# Autodesk Inventor assembly: DemonstratorUITräger
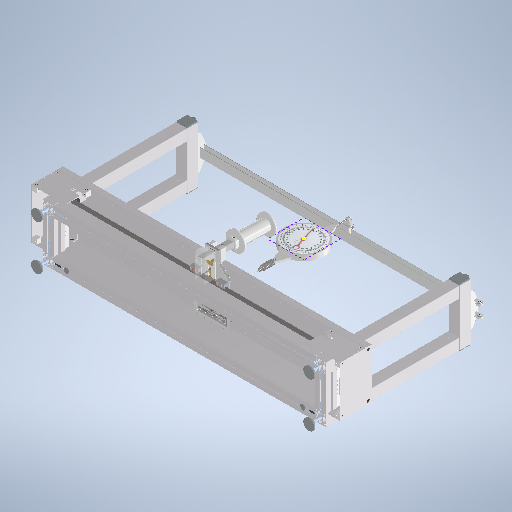
[picture p0: Inventor's stored thumbnail of the model, 512x512]
Saved by Autodesk Inventor 2025 (Build 290162010, 162A)
## iProperties
Created: 2024-11-07
Part Number: DemonstratorUITräger
Document SubType Name: Assembly
Designer: Admin
Mass: 19237.8 g
Surface Area: 46696.5 cm^2
Volume: 6430.49 cm^3
Density: 2.99166 g/cm^3
dummerWinkel: 1.5
Author: Admin
## Documents named in this file (39)
- C:\Users\Admin\GIT\HDVKBM\CAD\Krandemonstrator\DemonstratorUITräger.iam
- C:\Users\Admin\GIT\HDVKBM\CAD\Krandemonstrator\Träger.ipt
- C:\Users\Admin\GIT\HDVKBM\CAD\Krandemonstrator\Katze.iam
- C:\Users\Admin\GIT\HDVKBM\CAD\Krandemonstrator\UmlenkrolleHalterEinfach.iam
- C:\Users\Admin\GIT\HDVKBM\CAD\Krandemonstrator\SeilStange1m.ipt
- C:\Users\Admin\GIT\HDVKBM\CAD\Krandemonstrator\RollenhalterU.ipt
- C:\Users\Admin\GIT\HDVKBM\CAD\Krandemonstrator\UmlenkrolleHalterDoppelt.iam
- C:\Users\Admin\GIT\HDVKBM\CAD\Krandemonstrator\SeilatrappeHalter.ipt
- C:\Users\Admin\GIT\HDVKBM\CAD\Krandemonstrator\UmlenkrolleHalterDoppeltAngle.iam
- C:\Users\Admin\GIT\HDVKBM\CAD\Krandemonstrator\UmlenkrolleHalterEinfachAngle.iam
- C:\Users\Admin\GIT\HDVKBM\CAD\Krandemonstrator\UmlenkrolleHalterEinfachAngleB.iam
- C:\Users\Admin\GIT\HDVKBM\CAD\Krandemonstrator\seilatrappeHalterMini.ipt
- C:\Users\Admin\GIT\HDVKBM\CAD\Krandemonstrator\WS_10_40_930_2\WS_10_40_930_2.iam
- C:\Users\Admin\GIT\HDVKBM\CAD\Krandemonstrator\Frame.iam
- C:\Users\Admin\GIT\HDVKBM\CAD\Krandemonstrator\item_42006_nutenstein-8-st-m4-verzi__high\item_42006_nutenstein-8-st-m4-verzi__high.ipt
- C:\Users\Admin\GIT\HDVKBM\CAD\Krandemonstrator\item_2623_nutenstein-8-st-m6-verzi__high\item_2623_nutenstein-8-st-m6-verzi__high.ipt
- C:\Users\Admin\GIT\HDVKBM\CAD\Krandemonstrator\Zugfeder11.ipt
- C:\Users\Admin\GIT\HDVKBM\CAD\Krandemonstrator\Bedienhebel.iam
- C:\Users\Admin\GIT\HDVKBM\CAD\Krandemonstrator\SeilStange3cm.ipt
- C:\Users\Admin\GIT\HDVKBM\CAD\Krandemonstrator\waage.ipt
- C:\Users\Admin\GIT\HDVKBM\CAD\Krandemonstrator\verkleidungBremse.ipt
- C:\Users\Admin\Documents\Inventor\Content Center Files\R2025\de-DE\DIN EN ISO 7089\DIN EN ISO 7089 -  5.ipt
- C:\Users\Admin\Documents\Inventor\Content Center Files\R2025\de-DE\DIN 933\DIN 933 - M5  x 8.ipt
- C:\Users\Admin\GIT\HDVKBM\CAD\Krandemonstrator\item_42005_nutenstein-8-st-m5-verzi__high\item_42005_nutenstein-8-st-m5-verzi__high.ipt
- C:\Users\Admin\Documents\Inventor\Content Center Files\R2025\de-DE\DIN 933\DIN 933 - M5  x 18.ipt
- C:\Users\Admin\GIT\HDVKBM\CAD\Krandemonstrator\Schlitten.iam
- C:\Users\Admin\GIT\HDVKBM\CAD\Krandemonstrator\SeilStange447mm.ipt
- C:\Users\Admin\Documents\Inventor\Content Center Files\R2025\de-DE\ISO 4032(1)\ISO 4032 - M4DIN EN.ipt
- C:\Users\Admin\Documents\Inventor\Content Center Files\R2025\de-DE\DIN EN ISO 4026\DIN EN ISO 4026 - M4 x 8.ipt
- C:\Users\Admin\Documents\Inventor\Content Center Files\R2025\de-DE\ISO 2009(1)\ISO 2009 - M2 x 4 - DIN EN 2.ipt
- C:\Users\Admin\Documents\Inventor\Content Center Files\R2025\de-DE\ISO 10642(2)\ISO 10642  - M4  x  25.ipt
- C:\Users\Admin\Documents\Inventor\Content Center Files\R2025\de-DE\ISO 10642(2)\ISO 10642  - M6  x  16.ipt
- C:\Users\Admin\Documents\Inventor\Content Center Files\R2025\de-DE\ISO 10642(2)\ISO 10642  - M3  x  16.ipt
- C:\Users\Admin\Documents\Inventor\Content Center Files\R2025\de-DE\ISO 10642(2)\ISO 10642  - M3  x  25.ipt
- C:\Users\Admin\Documents\Inventor\Content Center Files\R2025\de-DE\ISO 2009(1)\ISO 2009 - M2 x 6 - DIN EN 4.ipt
- C:\Users\Admin\Documents\Inventor\Content Center Files\R2025\de-DE\ISO 10642(2)\ISO 10642  - M4  x  30.ipt
- C:\Users\Admin\GIT\HDVKBM\CAD\Krandemonstrator\Platte Scharfe Ecken (mm) 150 x 30 x 8 - UITräger.ipt
- C:\Users\Admin\GIT\HDVKBM\CAD\Krandemonstrator\MontageAufnahmeLO-LH_UI.ipt
- C:\Users\Admin\GIT\HDVKBM\CAD\Krandemonstrator\MontageAufnahmeLO_UI.ipt
## Components (139 placed, 40 different names)
1. Katze:1 [sub-assembly] — KatzeLagerHO, KatzeLagerVV, KatzeGewindeSeilStumpfVL, KatzeSeilStumpfHL, KatzeSeilStumpfVR, KatzeSeilStumpfHR, Zylindrisch:83
2. Frame:1 [sub-assembly] — Verschiebbar:90, Verschiebbar:89, Starr:89, Starr:124, Starr:134, Starr:136, Planar:60, Planar:61
3. DIN EN ISO 7089 5:1
4. DIN EN ISO 7089 5:2
5. DIN EN ISO 7089 5:3
6. DIN EN ISO 7089 5:4
7. DIN 933 - ersetzt durch DIN EN 24017 M5  x 8:1
8. DIN 933 - ersetzt durch DIN EN 24017 M5  x 8:2 — Zylindrisch:109
9. DIN 933 - ersetzt durch DIN EN 24017 M5  x 8:3
10. DIN 933 - ersetzt durch DIN EN 24017 M5  x 8:4 — Zylindrisch:110
11. Platte Scharfe Ecken (mm) 150 x 30 x 8 - UITräger:2 — Starr:136, Einfügen:8, Zylindrisch:110
12. Platte Scharfe Ecken (mm) 150 x 30 x 8 - UITräger:1 — Starr:134, Zylindrisch:109, Planar:57
13. DIN 933 - ersetzt durch DIN EN 24017 M5  x 18:2
14. DIN 933 - ersetzt durch DIN EN 24017 M5  x 18:3
15. DIN 933 - ersetzt durch DIN EN 24017 M5  x 18:4
16. DIN 933 - ersetzt durch DIN EN 24017 M5  x 18:1 — Einfügen:8
17. DIN EN ISO 10642 M3  x  25:1
18. DIN EN ISO 10642 M3  x  25:2
19. DIN EN ISO 10642 M3  x  25:3
20. DIN EN ISO 10642 M3  x  25:4
21. DIN EN ISO 10642 M3  x  16:1
22. DIN EN ISO 10642 M3  x  16:2
23. DIN EN ISO 10642 M3  x  16:3
24. DIN EN ISO 10642 M3  x  16:4
25. MontageAufnahmeLO-LH_UI:1 — SeilrolleORHplan, Starr:137
26. MontageAufnahmeLO_UI:1 — SeilrolleORVplan, Starr:138
27. MontageAufnahmeLOV:1 — SeilrolleOLVAuflage, Starr:140
28. MontageAufnahmeLOH:1 — SeilrolleOLHAuflage, Starr:139
29. item_42005_nutenstein-8-st-m5-verzi__high:1
30. item_42005_nutenstein-8-st-m5-verzi__high:2
31. item_42005_nutenstein-8-st-m5-verzi__high:4
32. item_42005_nutenstein-8-st-m5-verzi__high:3
33. Träger:1 — KatzeLagerHO, KatzeLagerVV, Starr:137, Starr:138, Starr:139, Starr:140, Planar:57
34. Bedienhebel:1 [sub-assembly] — Kugelförmig:1, Kugelförmig:3, Planar:58
35. DIN EN ISO 10642 M4  x  25:1
36. DIN EN ISO 10642 M4  x  25:2 — Zylindrisch:142
37. DIN EN ISO 10642 M4  x  25:3 — Zylindrisch:143
38. DIN EN ISO 10642 M4  x  25:4
39. verkleidungBremse:1 — Planar:59
40. DIN EN ISO 2009 M2 x 4:1
41. DIN EN ISO 2009 M2 x 4:2
42. DIN EN ISO 2009 M2 x 4:3
43. DIN EN ISO 2009 M2 x 4:4
44. Schlitten:1 [sub-assembly] — Zylindrisch:111, Zylindrisch:112, Zylindrisch:142, Zylindrisch:143, Planar:58, Planar:59, Verschiebbar:1, Kugelförmig:4, Kugelförmig:5
45. lastseil — Zylindrisch:83, Starr:117, Verschiebbar:1
46. Zugfeder1:1 — Starr:118
47. waage:1 — Starr:117, Starr:118
48. SeilStange3cm:5 — Zylindrisch:146, Kugelförmig:3
49. SeilStange3cm:6 — Zylindrisch:146, Kugelförmig:5
50. SeilStange3cm:7 — Starr:122
51. SeilStange3cm:8 — Starr:122, Starr:123
52. SeilStange3cm:2 — Zylindrisch:108, Kugelförmig:4
53. SeilStange3cm:1 — Kugelförmig:1, Zylindrisch:108, Starr:123
54. seilatrappeHalterMini:3 — SeilAtrappeHalterMini3, SeilAtrappeHalterMini3Seil
55. seilatrappeHalterMini:4 — SeilAtrappeHalterMini4, SeilAtrappeHalterMini4Seil
56. seilatrappeHalterMini:1 — SeilAtrappeHalterMini1, SeilAtrappeHalterMini1Seil
57. seilatrappeHalterMini:2 — SeilAtrappeHalterMini2, SeilAtrappeHalterMini2Seil
58. SeilatrappeHalter:1 — SeilAtrappeHalterSeilA, SeilAtrappeHalterSeilB, Starr:124
59. SeilStange1m:16 — SeilrolleULMVsld, SeilAtrappeHalterMini3Seil
60. SeilStange1m:17 — SeilrolleULMHsld, SeilAtrappeHalterMini4Seil
61. SeilStange1m:18 — SeilAtrappeHalterMini1Seil, SeilrolleORVver, SeilrolleURMVver
62. SeilStange1m:19 — SeilAtrappeHalterMini2Seil, SeilrolleORHver, SeilrolleURMHver
63. SeilStange1m:13 — SeilrolleURHsld
64. SeilStange1m:12 — SeilrolleURVsld
65. SeilStange1m:1 — KatzeGewindeSeilStumpfVL, SeilrolleOLVhor
66. SeilStange1m:3 — SeilrolleOLHhor, KatzeSeilStumpfHL
67. SeilStange1m:4 — SeilrolleORHhor, KatzeSeilStumpfHR
68. SeilStange1m:5 — SeilrolleORVhor, KatzeSeilStumpfVR
69. SeilStange1m:8 — SeilAtrappeHalterSeilB, SeilrolleOLHver, SeilrolleULHver
70. SeilStange1m:9 — SeilAtrappeHalterSeilA, SeilrolleOLVver, SeilrolleULVver
71. SeilStange1m:10 — Zylindrisch:15, SeilrolleULHhor, SeilrolleURHhor
72. SeilStange1m:11 — Zylindrisch:16, SeilrolleULVhor, SeilrolleURVhor
73. SeilStange1m:14 — SeilAtrappeRollenhalterSeilB, SeilrolleULMHhor, SeilrolleURMHhor
74. SeilStange1m:15 — SeilAtrappeRollenhalterSeilA, SeilrolleULMVhor, SeilrolleURMVhor
75. item_2623_nutenstein-8-st-m6-verzi__high:1 — Starr:90
76. item_2623_nutenstein-8-st-m6-verzi__high:2 — Starr:91
77. item_2623_nutenstein-8-st-m6-verzi__high:3 — Starr:96
78. item_2623_nutenstein-8-st-m6-verzi__high:4 — Starr:92
79. item_2623_nutenstein-8-st-m6-verzi__high:5 — Starr:93
80. item_2623_nutenstein-8-st-m6-verzi__high:6 — Starr:94
81. item_2623_nutenstein-8-st-m6-verzi__high:7 — Starr:95
82. item_2623_nutenstein-8-st-m6-verzi__high:8 — Starr:97
83. DIN EN ISO 10642 M6  x  16:1 — Starr:90, Starr:105
84. DIN EN ISO 10642 M6  x  16:2 — Starr:91, Starr:104
85. DIN EN ISO 10642 M6  x  16:3 — Starr:93, Starr:102
86. DIN EN ISO 10642 M6  x  16:4 — Starr:92, Starr:103
87. DIN EN ISO 10642 M6  x  16:5 — Starr:97, Starr:98
88. DIN EN ISO 10642 M6  x  16:6 — Starr:96, Starr:99
89. DIN EN ISO 10642 M6  x  16:7 — Starr:95, Starr:100
90. DIN EN ISO 10642 M6  x  16:8 — Starr:94, Starr:101
91. WS_10_40_930_2:1 [sub-assembly] — Starr:89, Zylindrisch:111, Zylindrisch:112, Starr:98, Starr:99, Starr:100, Starr:101, Starr:105, Starr:104, Starr:102, Starr:103
92. DIN EN ISO 2009 M2 x 6:1
93. DIN EN ISO 2009 M2 x 6:2
94. UmlenkrolleHalterEinfach:1 [sub-assembly] — SeilrolleOLVAuflage, SeilrolleOLVhor, SeilrolleOLVver
95. DIN EN ISO 2009 M2 x 6:3
96. DIN EN ISO 2009 M2 x 6:4
97. UmlenkrolleHalterEinfach:2 [sub-assembly] — SeilrolleOLHAuflage, SeilrolleOLHhor, SeilrolleOLHver
98. DIN EN 24032 M4:1
99. DIN EN 24032 M4:2
100. DIN EN 24032 M4:3
101. DIN EN 24032 M4:4
102. DIN EN ISO 4026 M4 x 8:1
103. DIN EN ISO 4026 M4 x 8:2
104. DIN EN ISO 4026 M4 x 8:3
105. DIN EN ISO 4026 M4 x 8:4
106. UmlenkrolleHalterEinfachAngle:1 [sub-assembly] — SeilrolleORVplan, SeilrolleORVhor, SeilrolleORVver, SeilAtrappeHalterMini1
107. DIN EN ISO 2009 M2 x 6:5
108. DIN EN ISO 2009 M2 x 6:6
109. DIN EN ISO 2009 M2 x 6:7
110. DIN EN ISO 2009 M2 x 6:8
111. UmlenkrolleHalterEinfachAngleB:1 [sub-assembly] — SeilrolleORHplan, SeilAtrappeHalterMini2, SeilrolleORHhor, SeilrolleORHver
112. RollenhalterU:1 — Planar:24, Planar:25, Planar:40, Zylindrisch:15, Zylindrisch:16, Starr:84, Starr:85, Verschiebbar:89, Planar:60
113. DIN EN ISO 10642 M4  x  30:1
114. DIN EN ISO 10642 M4  x  30:2
115. UmlenkrolleHalterDoppelt:1 [sub-assembly] — Planar:24, SeilrolleULMHhor, SeilrolleULMVhor, SeilrolleULMHsld, SeilrolleULMVsld, SeilAtrappeHalterMini3, SeilAtrappeHalterMini4
116. UmlenkrolleHalterEinfach:3 [sub-assembly] — Planar:25, SeilrolleULVver, SeilrolleULVhor
117. UmlenkrolleHalterEinfach:4 [sub-assembly] — Planar:40, SeilrolleULHver, SeilrolleULHhor
118. DIN EN ISO 2009 M2 x 6:9
119. DIN EN ISO 2009 M2 x 6:10
120. DIN EN ISO 2009 M2 x 6:11
121. DIN EN ISO 2009 M2 x 6:12
122. DIN EN ISO 2009 M2 x 6:13
123. item_42006_nutenstein-8-st-m4-verzi__high:1 — Starr:85
124. item_42006_nutenstein-8-st-m4-verzi__high:2 — Starr:84
125. DIN EN ISO 2009 M2 x 6:14
126. UmlenkrolleHalterEinfach:5 [sub-assembly] — Planar:42, SeilrolleURVhor, SeilrolleURVsld
127. UmlenkrolleHalterEinfach:6 [sub-assembly] — Planar:43, SeilrolleURHhor, SeilrolleURHsld
128. UmlenkrolleHalterDoppeltAngle:1 [sub-assembly] — Planar:54, SeilrolleURMHhor, SeilrolleURMVhor, SeilrolleURMVver, SeilrolleURMHver
129. DIN EN ISO 2009 M2 x 6:15
130. DIN EN ISO 2009 M2 x 6:16
131. DIN EN ISO 2009 M2 x 6:17
132. DIN EN ISO 2009 M2 x 6:18
133. DIN EN ISO 2009 M2 x 6:19
134. DIN EN ISO 2009 M2 x 6:20
135. RollenhalterU:2 — Planar:42, Planar:43, Planar:54, SeilAtrappeRollenhalterSeilB, SeilAtrappeRollenhalterSeilA, Verschiebbar:90, Starr:86, Starr:87, Planar:61
136. DIN EN ISO 10642 M4  x  30:3
137. item_42006_nutenstein-8-st-m4-verzi__high:3 — Starr:87
138. item_42006_nutenstein-8-st-m4-verzi__high:4 — Starr:86
139. DIN EN ISO 10642 M4  x  30:4
## Relationships (189: WeldJoint 74, CylindricalJoint 41, RelateRotateTranslate 24, Mate 18, PlanarJoint 17, Insert 8, BallJoint 4, TranslationJoint 3)
- KatzeLagerHO [PlanarJoint] (0.05 mm): Katze:1 ↔ Träger:1
- KatzeLagerVV [PlanarJoint] (0.05 mm): Katze:1 ↔ Träger:1
- [WeldJoint]: Katze:1 ↔ DIN EN 24032 M4:2
- [WeldJoint]: Katze:1 ↔ DIN EN 24032 M4:4
- [WeldJoint]: Katze:1 ↔ DIN EN 24032 M4:1
- [WeldJoint]: Katze:1 ↔ DIN EN 24032 M4:3
- KatzeGewindeSeilStumpfVL [WeldJoint]: Katze:1 ↔ SeilStange1m:1
- [WeldJoint]: Katze:1 ↔ DIN EN ISO 4026 M4 x 8:4
- [WeldJoint]: Katze:1 ↔ DIN EN ISO 4026 M4 x 8:2
- [WeldJoint]: Katze:1 ↔ DIN EN ISO 4026 M4 x 8:1
- [WeldJoint]: Katze:1 ↔ DIN EN ISO 4026 M4 x 8:3
- KatzeSeilStumpfHL [WeldJoint]: Katze:1 ↔ SeilStange1m:3
- KatzeSeilStumpfVR [WeldJoint]: Katze:1 ↔ SeilStange1m:5
- KatzeSeilStumpfHR [WeldJoint]: Katze:1 ↔ SeilStange1m:4
- [WeldJoint]: DIN EN ISO 2009 M2 x 6:2 ↔ UmlenkrolleHalterEinfach:1
- [WeldJoint]: DIN EN ISO 2009 M2 x 6:1 ↔ UmlenkrolleHalterEinfach:1
- SeilrolleOLVAuflage [PlanarJoint]: MontageAufnahmeLOV:1 ↔ UmlenkrolleHalterEinfach:1
- [CylindricalJoint]: MontageAufnahmeLOV:1 ↔ DIN EN ISO 2009 M2 x 6:1
- [CylindricalJoint]: MontageAufnahmeLOV:1 ↔ DIN EN ISO 2009 M2 x 6:2
- SeilrolleOLVhor [RelateRotateTranslate] (9 mm): SeilStange1m:1 ↔ UmlenkrolleHalterEinfach:1
- SeilrolleOLVver [RelateRotateTranslate] (9 mm): SeilStange1m:9 ↔ UmlenkrolleHalterEinfach:1
- [WeldJoint]: DIN EN ISO 2009 M2 x 6:3 ↔ UmlenkrolleHalterEinfach:2
- [WeldJoint]: DIN EN ISO 2009 M2 x 6:4 ↔ UmlenkrolleHalterEinfach:2
- SeilrolleOLHAuflage [PlanarJoint]: MontageAufnahmeLOH:1 ↔ UmlenkrolleHalterEinfach:2
- [CylindricalJoint]: MontageAufnahmeLOH:1 ↔ DIN EN ISO 2009 M2 x 6:3
- [CylindricalJoint]: MontageAufnahmeLOH:1 ↔ DIN EN ISO 2009 M2 x 6:4
- SeilrolleOLHhor [RelateRotateTranslate] (9 mm): SeilStange1m:3 ↔ UmlenkrolleHalterEinfach:2
- SeilrolleOLHver [RelateRotateTranslate] (9 mm): SeilStange1m:8 ↔ UmlenkrolleHalterEinfach:2
- Planar:24: RollenhalterU:1 ↔ UmlenkrolleHalterDoppelt:1
- [WeldJoint]: UmlenkrolleHalterDoppelt:1 ↔ DIN EN ISO 2009 M2 x 6:12
- [WeldJoint]: UmlenkrolleHalterDoppelt:1 ↔ DIN EN ISO 2009 M2 x 6:11
- [CylindricalJoint]: RollenhalterU:1 ↔ DIN EN ISO 2009 M2 x 6:12
- [CylindricalJoint]: RollenhalterU:1 ↔ DIN EN ISO 2009 M2 x 6:11
- [WeldJoint]: UmlenkrolleHalterEinfach:3 ↔ DIN EN ISO 2009 M2 x 6:13
- [WeldJoint]: UmlenkrolleHalterEinfach:3 ↔ DIN EN ISO 2009 M2 x 6:14
- Planar:25: RollenhalterU:1 ↔ UmlenkrolleHalterEinfach:3
- [CylindricalJoint]: RollenhalterU:1 ↔ DIN EN ISO 2009 M2 x 6:14
- [CylindricalJoint]: RollenhalterU:1 ↔ DIN EN ISO 2009 M2 x 6:13
- [WeldJoint]: UmlenkrolleHalterEinfach:4 ↔ DIN EN ISO 2009 M2 x 6:10
- [WeldJoint]: UmlenkrolleHalterEinfach:4 ↔ DIN EN ISO 2009 M2 x 6:9
- Planar:40: RollenhalterU:1 ↔ UmlenkrolleHalterEinfach:4
- [CylindricalJoint]: RollenhalterU:1 ↔ DIN EN ISO 2009 M2 x 6:9
- [CylindricalJoint]: RollenhalterU:1 ↔ DIN EN ISO 2009 M2 x 6:10
- SeilAtrappeHalterSeilA [CylindricalJoint]: SeilatrappeHalter:1 ↔ SeilStange1m:9
- SeilAtrappeHalterSeilB [CylindricalJoint]: SeilatrappeHalter:1 ↔ SeilStange1m:8
- Zylindrisch:15 [CylindricalJoint]: SeilStange1m:10 ↔ RollenhalterU:1
- Zylindrisch:16 [CylindricalJoint]: SeilStange1m:11 ↔ RollenhalterU:1
- SeilrolleULVver [RelateRotateTranslate] (9 mm): SeilStange1m:9 ↔ UmlenkrolleHalterEinfach:3
- SeilrolleULHver [RelateRotateTranslate] (9 mm): SeilStange1m:8 ↔ UmlenkrolleHalterEinfach:4
- SeilrolleULVhor [RelateRotateTranslate] (9 mm): SeilStange1m:11 ↔ UmlenkrolleHalterEinfach:3
- SeilrolleULHhor [RelateRotateTranslate] (9 mm): SeilStange1m:10 ↔ UmlenkrolleHalterEinfach:4
- [CylindricalJoint]: DIN EN ISO 2009 M2 x 6:19 ↔ RollenhalterU:2
- [CylindricalJoint]: DIN EN ISO 2009 M2 x 6:18 ↔ RollenhalterU:2
- [WeldJoint]: UmlenkrolleHalterEinfach:5 ↔ DIN EN ISO 2009 M2 x 6:17
- [WeldJoint]: UmlenkrolleHalterEinfach:5 ↔ DIN EN ISO 2009 M2 x 6:20
- Planar:42: UmlenkrolleHalterEinfach:5 ↔ RollenhalterU:2
- [CylindricalJoint]: DIN EN ISO 2009 M2 x 6:20 ↔ RollenhalterU:2
- [CylindricalJoint]: DIN EN ISO 2009 M2 x 6:17 ↔ RollenhalterU:2
- [WeldJoint]: UmlenkrolleHalterEinfach:6 ↔ DIN EN ISO 2009 M2 x 6:16
- [WeldJoint]: UmlenkrolleHalterEinfach:6 ↔ DIN EN ISO 2009 M2 x 6:15
- Planar:43: UmlenkrolleHalterEinfach:6 ↔ RollenhalterU:2
- [CylindricalJoint]: DIN EN ISO 2009 M2 x 6:16 ↔ RollenhalterU:2
- [CylindricalJoint]: DIN EN ISO 2009 M2 x 6:15 ↔ RollenhalterU:2
- SeilrolleURHhor [RelateRotateTranslate] (9 mm): SeilStange1m:10 ↔ UmlenkrolleHalterEinfach:6
- SeilrolleURVhor [RelateRotateTranslate] (9 mm): SeilStange1m:11 ↔ UmlenkrolleHalterEinfach:5
- SeilrolleURVsld [RelateRotateTranslate] (9 mm): SeilStange1m:12 ↔ UmlenkrolleHalterEinfach:5
- SeilrolleURHsld [RelateRotateTranslate] (9 mm): SeilStange1m:13 ↔ UmlenkrolleHalterEinfach:6
- Planar:54: UmlenkrolleHalterDoppeltAngle:1 ↔ RollenhalterU:2
- [WeldJoint]: UmlenkrolleHalterDoppeltAngle:1 ↔ DIN EN ISO 2009 M2 x 6:18
- [WeldJoint]: UmlenkrolleHalterDoppeltAngle:1 ↔ DIN EN ISO 2009 M2 x 6:19
- [WeldJoint]: UmlenkrolleHalterEinfachAngle:1 ↔ DIN EN ISO 2009 M2 x 6:6
- [WeldJoint]: UmlenkrolleHalterEinfachAngle:1 ↔ DIN EN ISO 2009 M2 x 6:5
- SeilrolleORVplan [PlanarJoint]: MontageAufnahmeLO_UI:1 ↔ UmlenkrolleHalterEinfachAngle:1
- [CylindricalJoint]: MontageAufnahmeLO_UI:1 ↔ DIN EN ISO 2009 M2 x 6:6
- [CylindricalJoint]: MontageAufnahmeLO_UI:1 ↔ DIN EN ISO 2009 M2 x 6:5
- [CylindricalJoint]: MontageAufnahmeLO-LH_UI:1 ↔ DIN EN ISO 2009 M2 x 6:8
- [CylindricalJoint]: MontageAufnahmeLO-LH_UI:1 ↔ DIN EN ISO 2009 M2 x 6:7
- SeilrolleORHplan [PlanarJoint]: MontageAufnahmeLO-LH_UI:1 ↔ UmlenkrolleHalterEinfachAngleB:1
- [WeldJoint]: DIN EN ISO 2009 M2 x 6:8 ↔ UmlenkrolleHalterEinfachAngleB:1
- [WeldJoint]: DIN EN ISO 2009 M2 x 6:7 ↔ UmlenkrolleHalterEinfachAngleB:1
- SeilAtrappeRollenhalterSeilB [CylindricalJoint]: SeilStange1m:14 ↔ RollenhalterU:2
- SeilAtrappeRollenhalterSeilA [CylindricalJoint]: SeilStange1m:15 ↔ RollenhalterU:2
- SeilrolleORHhor [RelateRotateTranslate] (9 mm): SeilStange1m:4 ↔ UmlenkrolleHalterEinfachAngleB:1
- SeilrolleORVhor [RelateRotateTranslate] (9 mm): SeilStange1m:5 ↔ UmlenkrolleHalterEinfachAngle:1
- SeilrolleORHver [RelateRotateTranslate] (9 mm): SeilStange1m:19 ↔ UmlenkrolleHalterEinfachAngleB:1
- SeilrolleORVver [RelateRotateTranslate] (9 mm): SeilStange1m:18 ↔ UmlenkrolleHalterEinfachAngle:1
- SeilrolleURMHhor [RelateRotateTranslate] (9 mm): SeilStange1m:14 ↔ UmlenkrolleHalterDoppeltAngle:1
- SeilrolleURMVhor [RelateRotateTranslate] (9 mm): SeilStange1m:15 ↔ UmlenkrolleHalterDoppeltAngle:1
- SeilrolleURMVver [RelateRotateTranslate] (9 mm): SeilStange1m:18 ↔ UmlenkrolleHalterDoppeltAngle:1
- SeilrolleURMHver [RelateRotateTranslate] (9 mm): SeilStange1m:19 ↔ UmlenkrolleHalterDoppeltAngle:1
- SeilrolleULMHhor [RelateRotateTranslate] (9 mm): SeilStange1m:14 ↔ UmlenkrolleHalterDoppelt:1
- SeilrolleULMVhor [RelateRotateTranslate] (9 mm): SeilStange1m:15 ↔ UmlenkrolleHalterDoppelt:1
- SeilrolleULMHsld [RelateRotateTranslate] (9 mm): SeilStange1m:17 ↔ UmlenkrolleHalterDoppelt:1
- SeilrolleULMVsld [RelateRotateTranslate] (9 mm): SeilStange1m:16 ↔ UmlenkrolleHalterDoppelt:1
- SeilAtrappeHalterMini1 [WeldJoint]: seilatrappeHalterMini:1 ↔ UmlenkrolleHalterEinfachAngle:1
- SeilAtrappeHalterMini1Seil [CylindricalJoint]: seilatrappeHalterMini:1 ↔ SeilStange1m:18
- SeilAtrappeHalterMini2 [WeldJoint]: seilatrappeHalterMini:2 ↔ UmlenkrolleHalterEinfachAngleB:1
- SeilAtrappeHalterMini2Seil [CylindricalJoint]: seilatrappeHalterMini:2 ↔ SeilStange1m:19
- SeilAtrappeHalterMini3 [WeldJoint]: seilatrappeHalterMini:3 ↔ UmlenkrolleHalterDoppelt:1
- SeilAtrappeHalterMini3Seil [CylindricalJoint]: seilatrappeHalterMini:3 ↔ SeilStange1m:16
- SeilAtrappeHalterMini4 [WeldJoint]: seilatrappeHalterMini:4 ↔ UmlenkrolleHalterDoppelt:1
- SeilAtrappeHalterMini4Seil [CylindricalJoint]: seilatrappeHalterMini:4 ↔ SeilStange1m:17
- Zylindrisch:83 [CylindricalJoint]: Katze:1 ↔ lastseil
- Verschiebbar:90 [TranslationJoint]: Frame:1 ↔ RollenhalterU:2
- Starr:84 [WeldJoint]: RollenhalterU:1 ↔ item_42006_nutenstein-8-st-m4-verzi__high:2
- Starr:85 [WeldJoint]: RollenhalterU:1 ↔ item_42006_nutenstein-8-st-m4-verzi__high:1
- [Mate]: RollenhalterU:1 ↔ DIN EN ISO 10642 M4  x  30:1
- [Mate]: RollenhalterU:1 ↔ DIN EN ISO 10642 M4  x  30:2
- [Mate]: RollenhalterU:2 ↔ DIN EN ISO 10642 M4  x  30:3
- [Mate]: RollenhalterU:2 ↔ DIN EN ISO 10642 M4  x  30:4
- Starr:86 [WeldJoint]: RollenhalterU:2 ↔ item_42006_nutenstein-8-st-m4-verzi__high:4
- Starr:87 [WeldJoint]: RollenhalterU:2 ↔ item_42006_nutenstein-8-st-m4-verzi__high:3
- Verschiebbar:89 [TranslationJoint]: Frame:1 ↔ RollenhalterU:1
- Starr:89 [WeldJoint] (1.5 mm): Frame:1 ↔ WS_10_40_930_2:1
- Starr:90 [WeldJoint]: item_2623_nutenstein-8-st-m6-verzi__high:1 ↔ DIN EN ISO 10642 M6  x  16:1
- Starr:91 [WeldJoint]: item_2623_nutenstein-8-st-m6-verzi__high:2 ↔ DIN EN ISO 10642 M6  x  16:2
- Starr:92 [WeldJoint]: item_2623_nutenstein-8-st-m6-verzi__high:4 ↔ DIN EN ISO 10642 M6  x  16:4
- Starr:93 [WeldJoint]: item_2623_nutenstein-8-st-m6-verzi__high:5 ↔ DIN EN ISO 10642 M6  x  16:3
- Starr:94 [WeldJoint]: item_2623_nutenstein-8-st-m6-verzi__high:6 ↔ DIN EN ISO 10642 M6  x  16:8
- Starr:95 [WeldJoint]: item_2623_nutenstein-8-st-m6-verzi__high:7 ↔ DIN EN ISO 10642 M6  x  16:7
- Starr:96 [WeldJoint]: item_2623_nutenstein-8-st-m6-verzi__high:3 ↔ DIN EN ISO 10642 M6  x  16:6
- Starr:97 [WeldJoint]: item_2623_nutenstein-8-st-m6-verzi__high:8 ↔ DIN EN ISO 10642 M6  x  16:5
- Starr:98 [WeldJoint]: DIN EN ISO 10642 M6  x  16:5 ↔ WS_10_40_930_2:1
- Starr:99 [WeldJoint]: DIN EN ISO 10642 M6  x  16:6 ↔ WS_10_40_930_2:1
- Starr:100 [WeldJoint]: DIN EN ISO 10642 M6  x  16:7 ↔ WS_10_40_930_2:1
- Starr:101 [WeldJoint]: DIN EN ISO 10642 M6  x  16:8 ↔ WS_10_40_930_2:1
- Starr:102 [WeldJoint]: DIN EN ISO 10642 M6  x  16:3 ↔ WS_10_40_930_2:1
- Starr:103 [WeldJoint]: DIN EN ISO 10642 M6  x  16:4 ↔ WS_10_40_930_2:1
- Starr:104 [WeldJoint]: DIN EN ISO 10642 M6  x  16:2 ↔ WS_10_40_930_2:1
- Starr:105 [WeldJoint]: DIN EN ISO 10642 M6  x  16:1 ↔ WS_10_40_930_2:1
- [Mate]: Bedienhebel:1 ↔ DIN EN ISO 10642 M4  x  25:1
- [Mate]: Bedienhebel:1 ↔ DIN EN ISO 10642 M4  x  25:2
- [Mate]: Bedienhebel:1 ↔ DIN EN ISO 10642 M4  x  25:3
- [Mate]: Bedienhebel:1 ↔ DIN EN ISO 10642 M4  x  25:4
- Zylindrisch:108 [CylindricalJoint]: SeilStange3cm:2 ↔ SeilStange3cm:1
- Kugelförmig:1 [BallJoint]: Bedienhebel:1 ↔ SeilStange3cm:1
- Starr:117 [WeldJoint] (-430 mm): lastseil ↔ waage:1
- Starr:118 [WeldJoint]: Zugfeder1:1 ↔ waage:1
- Zylindrisch:146 [CylindricalJoint]: SeilStange3cm:5 ↔ SeilStange3cm:6
- Kugelförmig:3 [BallJoint]: Bedienhebel:1 ↔ SeilStange3cm:5
- Starr:122 [WeldJoint]: SeilStange3cm:7 ↔ SeilStange3cm:8
- Starr:123 [WeldJoint]: SeilStange3cm:8 ↔ SeilStange3cm:1
- Starr:124 [WeldJoint]: Frame:1 ↔ SeilatrappeHalter:1
- [Mate]: verkleidungBremse:1 ↔ DIN EN ISO 2009 M2 x 4:1
- [Mate]: verkleidungBremse:1 ↔ DIN EN ISO 2009 M2 x 4:2
- [WeldJoint]: DIN EN ISO 7089 5:1 ↔ Träger:1
- [WeldJoint]: DIN EN ISO 7089 5:2 ↔ Träger:1
- [WeldJoint]: DIN EN ISO 7089 5:4 ↔ Träger:1
- [WeldJoint]: DIN EN ISO 7089 5:3 ↔ Träger:1
- Starr:134 [WeldJoint]: Frame:1 ↔ Platte Scharfe Ecken (mm) 150 x 30 x 8 - UITräger:1
- [Insert]: DIN EN ISO 7089 5:3 ↔ DIN 933 - ersetzt durch DIN EN 24017 M5  x 8:1
- [Insert]: DIN EN ISO 7089 5:4 ↔ DIN 933 - ersetzt durch DIN EN 24017 M5  x 8:2
- [Insert]: DIN EN ISO 7089 5:2 ↔ DIN 933 - ersetzt durch DIN EN 24017 M5  x 8:3
- [Insert]: DIN EN ISO 7089 5:1 ↔ DIN 933 - ersetzt durch DIN EN 24017 M5  x 8:4
- Starr:136 [WeldJoint]: Frame:1 ↔ Platte Scharfe Ecken (mm) 150 x 30 x 8 - UITräger:2
- [Insert]: Platte Scharfe Ecken (mm) 150 x 30 x 8 - UITräger:1 ↔ DIN 933 - ersetzt durch DIN EN 24017 M5  x 18:2
- [Insert]: Platte Scharfe Ecken (mm) 150 x 30 x 8 - UITräger:1 ↔ DIN 933 - ersetzt durch DIN EN 24017 M5  x 18:3
- [Insert]: Platte Scharfe Ecken (mm) 150 x 30 x 8 - UITräger:2 ↔ DIN 933 - ersetzt durch DIN EN 24017 M5  x 18:4
- Einfügen:8 [Insert]: Platte Scharfe Ecken (mm) 150 x 30 x 8 - UITräger:2 ↔ DIN 933 - ersetzt durch DIN EN 24017 M5  x 18:1
- Starr:137 [WeldJoint]: MontageAufnahmeLO-LH_UI:1 ↔ Träger:1
- Starr:138 [WeldJoint]: MontageAufnahmeLO_UI:1 ↔ Träger:1
- Starr:139 [WeldJoint]: MontageAufnahmeLOH:1 ↔ Träger:1
- Starr:140 [WeldJoint]: MontageAufnahmeLOV:1 ↔ Träger:1
- [Mate]: DIN EN ISO 10642 M3  x  16:1 ↔ MontageAufnahmeLOH:1
- [Mate]: DIN EN ISO 10642 M3  x  25:1 ↔ MontageAufnahmeLOH:1
- [Mate]: DIN EN ISO 10642 M3  x  25:2 ↔ MontageAufnahmeLOV:1
- [Mate]: DIN EN ISO 10642 M3  x  16:2 ↔ MontageAufnahmeLOV:1
- [Mate]: DIN EN ISO 10642 M3  x  16:3 ↔ MontageAufnahmeLO-LH_UI:1
- [Mate]: DIN EN ISO 10642 M3  x  25:3 ↔ MontageAufnahmeLO-LH_UI:1
- [Mate]: DIN EN ISO 10642 M3  x  16:4 ↔ MontageAufnahmeLO_UI:1
- [Mate]: DIN EN ISO 10642 M3  x  25:4 ↔ MontageAufnahmeLO_UI:1
- Zylindrisch:109 [CylindricalJoint]: DIN 933 - ersetzt durch DIN EN 24017 M5  x 8:2 ↔ Platte Scharfe Ecken (mm) 150 x 30 x 8 - UITräger:1
- Planar:57: Platte Scharfe Ecken (mm) 150 x 30 x 8 - UITräger:1 ↔ Träger:1
- Zylindrisch:110 [CylindricalJoint]: DIN 933 - ersetzt durch DIN EN 24017 M5  x 8:4 ↔ Platte Scharfe Ecken (mm) 150 x 30 x 8 - UITräger:2
- Zylindrisch:111 [CylindricalJoint]: Schlitten:1 ↔ WS_10_40_930_2:1
- Zylindrisch:112 [CylindricalJoint]: Schlitten:1 ↔ WS_10_40_930_2:1
- Zylindrisch:142 [CylindricalJoint]: DIN EN ISO 10642 M4  x  25:2 ↔ Schlitten:1
- Zylindrisch:143 [CylindricalJoint]: DIN EN ISO 10642 M4  x  25:3 ↔ Schlitten:1
- Planar:58: Bedienhebel:1 ↔ Schlitten:1
- Planar:59: verkleidungBremse:1 ↔ Schlitten:1
- [CylindricalJoint]: DIN EN ISO 2009 M2 x 4:1 ↔ Schlitten:1
- [CylindricalJoint]: DIN EN ISO 2009 M2 x 4:2 ↔ Schlitten:1
- [WeldJoint]: DIN EN ISO 2009 M2 x 4:4 ↔ Schlitten:1
- [WeldJoint]: DIN EN ISO 2009 M2 x 4:3 ↔ Schlitten:1
- Verschiebbar:1 [TranslationJoint]: Schlitten:1 ↔ lastseil
- Kugelförmig:4 [BallJoint]: Schlitten:1 ↔ SeilStange3cm:2
- Kugelförmig:5 [BallJoint]: Schlitten:1 ↔ SeilStange3cm:6
- Planar:60 (-6 mm): Frame:1 ↔ RollenhalterU:1
- Planar:61 (-6 mm): Frame:1 ↔ RollenhalterU:2
## Named parameters: Finish2_Area = 2050.01, Finish4_Area = 0.0628319
note: some values were not read from the file. Shown as the stored number, unit unknown: "Finish2_Area", "Finish4_Area".
